# Autodesk Inventor assembly: 回路全部
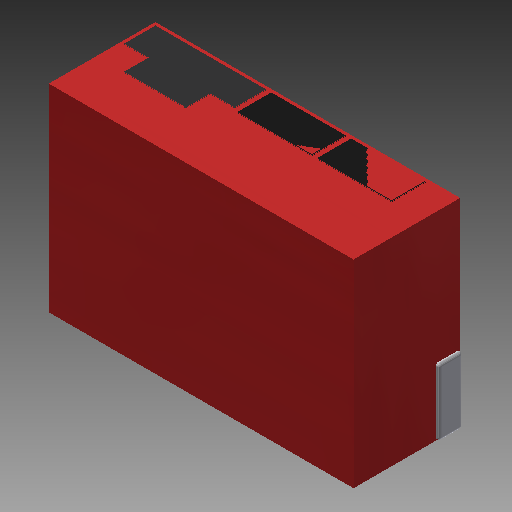
[picture p0: Inventor's stored thumbnail of the model, 512x512]
Saved by Autodesk Inventor 2019 (Build 230136000, 136)
## iProperties
Part Number: 回路全部
Material: 一般
Document SubType Name: Assembly
Designer: 雪村
Mass: 185.5 g
Surface Area: 493.771 cm^2
Volume: 282.889 cm^3
Density: 0.655735 g/cm^3
Author: 雪村
## Documents named in this file (3)
- C:\Users\white\Documents\SRDC\SRDC\Inventor_2017\2018年機体\2018年2年機体　雪村\回路全部.iam
- C:\Users\white\Documents\SRDC\SRDC\Inventor_2017\2018年機体\2018年2年機体　雪村\回路.中身.iam
- C:\Users\white\Documents\SRDC\SRDC\Inventor_2017\2018年機体\2018年2年機体　雪村\回路2.ipt
## Components (2 placed, 2 different names)
1. 回路.中身:1 [sub-assembly] — フラッシュ:1, フラッシュ:2, フラッシュ:3
2. 回路2:1 — フラッシュ:1, フラッシュ:2, フラッシュ:3
## Relationships (3: Flush 3)
- フラッシュ:1 [Flush]: 回路.中身:1 ↔ 回路2:1
- フラッシュ:2 [Flush]: 回路.中身:1 ↔ 回路2:1
- フラッシュ:3 [Flush]: 回路.中身:1 ↔ 回路2:1
